# Autodesk Inventor assembly: mppcInterface
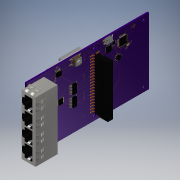
[picture p0: Inventor's stored thumbnail of the model, 180x180]
Saved by Autodesk Inventor 2016 (Build 200138000, 138)
## iProperties
Created: 2016-04-06
Part Number: mppcInterface
Document SubType Name: Assembly
Designer: sawai
Author: sawai
## Documents named in this file (17)
- C:\Users\Jonathan\Documents\Projects\mppcInterface\4-channel\mppcInterface\cad\mppcInterface.iam
- C:\Users\Jonathan\Documents\Projects\mppcInterface\4-channel\mppcInterface\cad\mppcInterfacePcb.ipt
- C:\Users\Jonathan\Documents\Projects\mppcInterface\4-channel\mppcInterface\cad\connector\SS-668804S-A-PG4-AC.ipt
- C:\Users\Jonathan\Documents\Projects\mppcInterface\4-channel\mppcInterface\cad\electronics\DX4R005H91.ipt
- C:\Users\Jonathan\Documents\Projects\mppcInterface\4-channel\mppcInterface\cad\electronics\FSM2JSMAA.ipt
- C:\Users\Jonathan\Documents\Projects\mppcInterface\4-channel\mppcInterface\cad\electronics\32 TQFP.ipt
- C:\Users\Jonathan\Documents\Projects\mppcInterface\4-channel\mppcInterface\cad\electronics\403C.ipt
- C:\Users\Jonathan\Documents\Projects\mppcInterface\4-channel\mppcInterface\cad\electronics\LXDC2HN18A-097.ipt
- C:\Users\Jonathan\Documents\Projects\mppcInterface\4-channel\mppcInterface\cad\electronics\VQFN.ipt
- C:\Users\Jonathan\Documents\Projects\mppcInterface\4-channel\mppcInterface\cad\electronics\QFN-28.ipt
- C:\Users\Jonathan\Documents\Projects\mppcInterface\4-channel\mppcInterface\cad\electronics\soic-8-N.ipt
- C:\Users\Jonathan\Documents\Projects\anodePiShield\coincidenceCounter\cad\electronics\soic\soic.ipt
- C:\Users\Jonathan\Documents\Projects\mppcInterface\4-channel\mppcInterface\cad\electronics\soic-14-N.ipt
- C:\Users\Jonathan\Documents\Projects\nonmodular\coincidenceCounter\cad\electronics\soic\soic.ipt
- C:\Users\Jonathan\Documents\Projects\mppcInterface\4-channel\mppcInterface\cad\connector\SMT GPIO Female Header 2x20\assembly.iam
- C:\Users\Jonathan\Documents\Projects\mppcInterface\4-channel\mppcInterface\cad\electronics\TSSOP.ipt
- C:\Users\Jonathan\Documents\Projects\mppcHighVoltage\mppcHighVoltage\cad\highVoltageMppcBoard.iam
## Components (18 placed, 14 different names)
1. mppcInterfacePcb:1 — Mate:1, Angle:1, Mate:2, Angle:2, Mate:3, Angle:3, Mate:4, Angle:4, Mate:5, Angle:5, Mate:6, Angle:6, Mate:7, Angle:7, Mate:8, Angle:8, Mate:9, Angle:9, Mate:10, Angle:10, Mate:11, Angle:11, Mate:12, Angle:12, Mate:13, Angle:13
2. SS-668804S-A-PG4-AC:1 — Mate:1, Angle:1
3. DX4R005H91:1 — Mate:2, Angle:2
4. FSM2JSMAA:1 — Mate:3, Angle:3
5. 32 TQFP:1 — Mate:4, Angle:4
6. 403C:1 — Mate:5, Angle:5
7. LXDC2HN18A-097:1 — Mate:6, Angle:6
8. VQFN:1 — Mate:7, Angle:7
9. QFN-28:1 — Mate:8, Angle:8
10. soic-8-N:1 — Mate:9, Angle:9
11. soic-14-N:2 — Flush:1, Flush:2, Mate:10
12. soic-14-N:3 — Flush:1, Flush:2, Angle:10
13. assembly:1 [sub-assembly] — Mate:11, Angle:11
14. TSSOP:1 — Mate:12, Angle:12
15. highVoltageMppcBoard:1 [sub-assembly] — Mate:13, Angle:13
16. highVoltageMppcBoard:2 [sub-assembly]
17. highVoltageMppcBoard:3 [sub-assembly]
18. highVoltageMppcBoard:4 [sub-assembly]
## Component patterns: (4 elements, first: highVoltageMppcBoard:1)
## Relationships (28: Mate 13, Angle 13, Flush 2)
- Mate:1: mppcInterfacePcb:1 ↔ SS-668804S-A-PG4-AC:1
- Angle:1 (0 deg): mppcInterfacePcb:1 ↔ SS-668804S-A-PG4-AC:1
- Mate:2: mppcInterfacePcb:1 ↔ DX4R005H91:1
- Angle:2 (0 deg): mppcInterfacePcb:1 ↔ DX4R005H91:1
- Mate:3: mppcInterfacePcb:1 ↔ FSM2JSMAA:1
- Angle:3 (0 deg): mppcInterfacePcb:1 ↔ FSM2JSMAA:1
- Mate:4: mppcInterfacePcb:1 ↔ 32 TQFP:1
- Angle:4 (0 deg): mppcInterfacePcb:1 ↔ 32 TQFP:1
- Mate:5: mppcInterfacePcb:1 ↔ 403C:1
- Angle:5 (0 deg): mppcInterfacePcb:1 ↔ 403C:1
- Mate:6: mppcInterfacePcb:1 ↔ LXDC2HN18A-097:1
- Angle:6 (0 deg): mppcInterfacePcb:1 ↔ LXDC2HN18A-097:1
- Mate:7: mppcInterfacePcb:1 ↔ VQFN:1
- Angle:7 (135 deg): mppcInterfacePcb:1 ↔ VQFN:1
- Mate:8: mppcInterfacePcb:1 ↔ QFN-28:1
- Angle:8 (0 deg): mppcInterfacePcb:1 ↔ QFN-28:1
- Mate:9: mppcInterfacePcb:1 ↔ soic-8-N:1
- Angle:9 (0 deg): mppcInterfacePcb:1 ↔ soic-8-N:1
- Flush:1: soic-14-N:2 ↔ soic-14-N:3
- Flush:2: soic-14-N:2 ↔ soic-14-N:3
- Mate:10: mppcInterfacePcb:1 ↔ soic-14-N:2
- Angle:10 (0 deg): mppcInterfacePcb:1 ↔ soic-14-N:3
- Mate:11: mppcInterfacePcb:1 ↔ assembly:1
- Angle:11 (0 deg): mppcInterfacePcb:1 ↔ assembly:1
- Mate:12: mppcInterfacePcb:1 ↔ TSSOP:1
- Angle:12 (0 deg): mppcInterfacePcb:1 ↔ TSSOP:1
- Mate:13: mppcInterfacePcb:1 ↔ highVoltageMppcBoard:1
- Angle:13 (0 deg): mppcInterfacePcb:1 ↔ highVoltageMppcBoard:1
